# Autodesk Inventor assembly: Motor V4
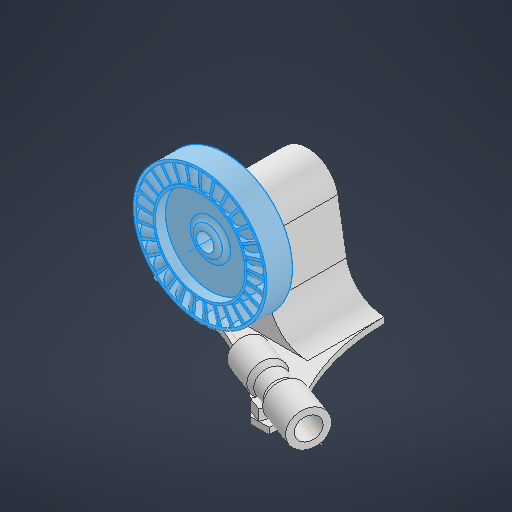
[picture p0: Inventor's stored thumbnail of the model, 512x512]
Saved by Autodesk Inventor 2025.3 (Build 293356030, 356C)
## iProperties
Created: 2025-09-22
Part Number: Motor V4
Document SubType Name: Assembly
Designer: yo
Author: yo
## Documents named in this file (4)
- C:\Users\yo\Documents\Andes\9no Semestre\Proyecto Intermedio\Proyecto\Huron-Hudson\Versions\V4\Motor V4.iam
- C:\Users\yo\Documents\Andes\9no Semestre\Proyecto Intermedio\Proyecto\Huron-Hudson\Versions\V4\Support.ipt
- C:\Users\yo\Documents\Andes\9no Semestre\Proyecto Intermedio\Proyecto\Huron-Hudson\Versions\V2\Pelton - V2.ipt
- C:\Users\yo\Documents\Andes\9no Semestre\Proyecto Intermedio\Proyecto\Huron-Hudson\Versions\V2\Reductor.ipt
## Components (3 placed, 3 different names)
1. Support:1 — Flush:1, Flush:2, Flush:3, Mate:3, Mate:4, Mate:5, Mate:6
2. Pelton - V2:1 — Mate:6
3. Reductor:1 — Mate:3, Mate:4, Mate:5
## Relationships (7: Mate 4, Flush 3)
- Flush:1: Support:1
- Flush:2: Support:1
- Flush:3: Support:1
- Mate:3: Support:1 ↔ Reductor:1
- Mate:4: Support:1 ↔ Reductor:1
- Mate:5: Support:1 ↔ Reductor:1
- Mate:6: Support:1 ↔ Pelton - V2:1
